# Autodesk Inventor assembly: 조립품4
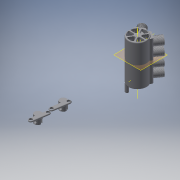
[picture p0: Inventor's stored thumbnail of the model, 180x180]
Saved by Autodesk Inventor 2018 (Build 220112000, 112)
## iProperties
Created: 2019-05-28
Part Number: 조립품4
Material: 일반
Document SubType Name: Assembly
Designer: LeeYounSeo
Author: LeeYounSeo
## Documents named in this file (5)
- C:\Users\LeeYounSeo\Desktop\조립품4.iam
- C:\Users\LeeYounSeo\Desktop\새 폴더 (2)\부품2.ipt
- C:\Users\LeeYounSeo\Desktop\새 폴더 (2)\부품3.ipt
- C:\Users\LeeYounSeo\Desktop\새 폴더 (2)\부품4.ipt
- C:\Users\LeeYounSeo\Desktop\새 폴더 (2)\부품7.ipt
## Components (6 placed, 4 different names)
1. 부품2:1 — 메이트:1, 플러쉬:1
2. 부품3:1 — 메이트:1, 플러쉬:1
3. 부품4:1
4. 부품4:2
5. 부품7:1
6. 부품7:2
## Relationships (2: Mate 1, Flush 1)
- 메이트:1 [Mate]: 부품2:1 ↔ 부품3:1
- 플러쉬:1 [Flush]: 부품2:1 ↔ 부품3:1
